# Autodesk Inventor assembly: BiasTee
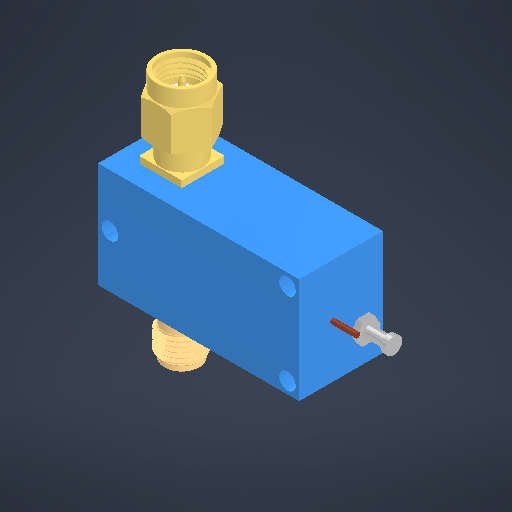
[picture p0: Inventor's stored thumbnail of the model, 512x512]
Saved by Autodesk Inventor 2026.2 (Build 302298010, 298A)
## iProperties
Created: 2026-06-12
Part Number: BiasTee
Document SubType Name: Assembly
Designer: sonata
Author: sonata
## Documents named in this file (4)
- Z:\crush\BiasTee.iam
- Z:\crush\BTBody.ipt
- Z:\crush\crush\sma-female-pcb-edge-launch-connector-031-pcb-thickness-1.snapshot.1\2985-6037\2985-6037\2985-6037.ipt
- Z:\crush\sma-male-edge-mount-1.snapshot.4\SMA_male_edge_6.5x6.5\SMA_male_edge_6.5x6.5\SMA_male_edge_6.5x6.5.ipt
## Components (3 placed, 3 different names)
1. BTBody:1 — Mate:1, Flush:2, Flush:3, Mate:2, Flush:4, Flush:5
2. 2985-6037:1 — Mate:1, Flush:2, Flush:3
3. SMA_male_edge_6.5x6.5:1 — Mate:2, Flush:4, Flush:5
## Relationships (6: Flush 4, Mate 2)
- Mate:1: BTBody:1 ↔ 2985-6037:1
- Flush:2 (2.3876 mm): BTBody:1 ↔ 2985-6037:1
- Flush:3 (1.5748 mm): BTBody:1 ↔ 2985-6037:1
- Mate:2 (-0.508 mm): BTBody:1 ↔ SMA_male_edge_6.5x6.5:1
- Flush:4 (3.0988 mm): BTBody:1 ↔ SMA_male_edge_6.5x6.5:1
- Flush:5 (3.0988 mm): BTBody:1 ↔ SMA_male_edge_6.5x6.5:1
